# Autodesk Inventor assembly: Hand Assembly
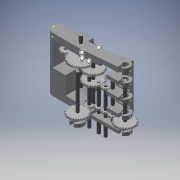
[picture p0: Inventor's stored thumbnail of the model, 180x180]
Saved by Autodesk Inventor 2017 (Build 210142000, 142)
## iProperties
Created: 2016-09-28
Part Number: Hand Assembly
Document SubType Name: Assembly
Designer: cmcdona
Author: cmcdona
## Documents named in this file (28)
- D:\julie\Documents\Cours McMaster\Graphics & Design\Project\Hand Assembly.iam
- D:\julie\Documents\Cours McMaster\Graphics & Design\Project\Hand - Frame.ipt
- D:\julie\Documents\Cours McMaster\Graphics & Design\Project\Hand - Digit 4.ipt
- D:\julie\Documents\Cours McMaster\Graphics & Design\Project\Hand - Digit 0-1.ipt
- D:\julie\Documents\Cours McMaster\Graphics & Design\Project\Hand - Distal Bridge.ipt
- D:\julie\Documents\Cours McMaster\Graphics & Design\Project\Hand - Digit 2-3.ipt
- D:\julie\Documents\Cours McMaster\Graphics & Design\Project\Hand - Proximal Bridge.ipt
- D:\julie\Documents\Cours McMaster\Graphics & Design\Project\Hand - Functional Workspace.ipt
- D:\julie\Documents\Cours McMaster\Graphics & Design\Project\Input Motor.ipt
- D:\julie\Documents\Cours McMaster\Graphics & Design\Project\Forefingers Rod.ipt
- D:\julie\Documents\Cours McMaster\Graphics & Design\Project\Hand Assembly\Design Accelerator\Spur Gears3.iam
- D:\julie\Documents\Cours McMaster\Graphics & Design\Project\Hand Assembly\Design Accelerator\Spur Gears4.iam
- D:\julie\Documents\Cours McMaster\Graphics & Design\Project\Hand Assembly\Design Accelerator\Spur Gears5.iam
- D:\julie\Documents\Cours McMaster\Graphics & Design\Project\Hand Assembly\Design Accelerator\Spur Gears6.iam
- D:\julie\Documents\Cours McMaster\Graphics & Design\Project\Hand Assembly\Design Accelerator\Spur Gear13.ipt
- D:\julie\Documents\Cours McMaster\Graphics & Design\Project\Hand Assembly\Design Accelerator\Spur Gear23.ipt
- D:\julie\Documents\Cours McMaster\Graphics & Design\Project\Hand Assembly\Design Accelerator\Spur Gear14.ipt
- D:\julie\Documents\Cours McMaster\Graphics & Design\Project\Hand Assembly\Design Accelerator\Spur Gear24.ipt
- D:\julie\Documents\Cours McMaster\Graphics & Design\Project\Hand Assembly\Design Accelerator\Spur Gear15.ipt
- D:\julie\Documents\Cours McMaster\Graphics & Design\Project\Hand Assembly\Design Accelerator\Spur Gear25.ipt
- D:\julie\Documents\Cours McMaster\Graphics & Design\Project\Hand Assembly\Design Accelerator\Spur Gear16.ipt
- D:\julie\Documents\Cours McMaster\Graphics & Design\Project\Hand Assembly\Design Accelerator\Spur Gear26.ipt
- D:\julie\Documents\Cours McMaster\Graphics & Design\Project\Hand Assembly\Design Accelerator\Spur Gears8.iam
- D:\julie\Documents\Cours McMaster\Graphics & Design\Project\Hand Assembly\Design Accelerator\Spur Gears9.iam
- D:\julie\Documents\Cours McMaster\Graphics & Design\Project\Hand Assembly\Design Accelerator\Spur Gear18.ipt
- D:\julie\Documents\Cours McMaster\Graphics & Design\Project\Hand Assembly\Design Accelerator\Spur Gear28.ipt
- D:\julie\Documents\Cours McMaster\Graphics & Design\Project\Hand Assembly\Design Accelerator\Spur Gear19.ipt
- D:\julie\Documents\Cours McMaster\Graphics & Design\Project\Hand Assembly\Design Accelerator\Spur Gear29.ipt
## Components (40 placed, 12 different names)
1. Hand - Frame:1 — Flush:1, Flush:2, Mate:1, Mate:2, Flush:3, Mate:3, Mate:16, Mate:17, Mate:18, Mate:22, Mate:23, Mate:25
2. Hand - Digit 4:1 — Flush:1, Flush:2, Mate:1, Mate:4, Mate:5, Mate:24
3. Hand - Digit 0-1:1 — Mate:2, Flush:3, Mate:3, Mate:6, Mate:19, Mate:20, Mate:21, Flush:4, Mate:37, Flush:23
4. Hand - Distal Bridge:1 — Mate:4, Mate:5, Mate:6, Mate:7, Mate:8, Mate:9, Mate:10, Mate:11, Mate:12, Mate:13, Mate:14, Mate:15
5. Hand - Digit 2-3:1 — Mate:7, Mate:8, Mate:9
6. Hand - Digit 2-3:2 — Mate:10, Mate:11, Mate:12
7. Hand - Digit 2-3:3 — Mate:13, Mate:14, Mate:15
8. Hand - Proximal Bridge:1 — Mate:16, Mate:17, Mate:18
9. Hand - Functional Workspace:1 — Mate:19, Mate:20, Mate:21
10. Input Motor:1 — Mate:22, Mate:23, Mate:25
11. Forefingers Rod:1 — Mate:24, Flush:4, Mate:26, Mate:27, Angle:1
12. Spur Gears:1 [sub-assembly]
13. Spur Gears:2 [sub-assembly]
14. Spur Gears:3 [sub-assembly]
15. Spur Gears:4 [sub-assembly]
16. Spur Gear1:1 — Mate:26, Flush:5
17. Spur Gear2:1 — Flush:5, Flush:6, Angle:1, Flush:10, Mate:39
18. Spur Gear1:2 — Flush:9, Flush:11, Mate:42
19. Spur Gear2:2 — Flush:9, Flush:11, Mate:41
20. Spur Gear1:3 — Flush:14, Mate:43
21. Spur Gear2:3 — Flush:14, Mate:36, Mate:44
22. Spur Gear1:4 — Mate:36, Flush:16, Mate:45
23. Spur Gear2:4 — Flush:16
24. Spur Gears:6 [sub-assembly]
25. Spur Gears:7 [sub-assembly]
26. Spur Gear1:5 — Flush:19
27. Spur Gear2:6 — Flush:18, Flush:19
28. Spur Gear1:6 — Flush:17, Flush:18
29. Spur Gear2:7 — Mate:27, Flush:17
30. Spur Gear2:8 — Flush:6, Flush:10, Flush:20, Flush:21, Mate:40
31. Spur Gear1:7 — Flush:20, Mate:38
32. Spur Gear2:9 — Flush:21, Flush:22, Mate:46
33. Spur Gear2:10 — Flush:22, Mate:47
34. Forefingers Rod:2 — Mate:39
35. Forefingers Rod:3 — Mate:37, Flush:23, Mate:38
36. Forefingers Rod:4 — Mate:40, Mate:41
37. Forefingers Rod:5 — Mate:42, Mate:43
38. Forefingers Rod:6 — Mate:44, Mate:45
39. Forefingers Rod:7 — Mate:46
40. Forefingers Rod:8 — Mate:47
## Relationships (58: Mate 39, Flush 18, Angle 1)
- Flush:1: Hand - Frame:1 ↔ Hand - Digit 4:1
- Flush:2: Hand - Frame:1 ↔ Hand - Digit 4:1
- Mate:1: Hand - Frame:1 ↔ Hand - Digit 4:1
- Mate:2: Hand - Frame:1 ↔ Hand - Digit 0-1:1
- Flush:3: Hand - Frame:1 ↔ Hand - Digit 0-1:1
- Mate:3: Hand - Frame:1 ↔ Hand - Digit 0-1:1
- Mate:4: Hand - Digit 4:1 ↔ Hand - Distal Bridge:1
- Mate:5: Hand - Digit 4:1 ↔ Hand - Distal Bridge:1
- Mate:6: Hand - Digit 0-1:1 ↔ Hand - Distal Bridge:1
- Mate:7: Hand - Distal Bridge:1 ↔ Hand - Digit 2-3:1
- Mate:8: Hand - Distal Bridge:1 ↔ Hand - Digit 2-3:1
- Mate:9: Hand - Distal Bridge:1 ↔ Hand - Digit 2-3:1
- Mate:10: Hand - Distal Bridge:1 ↔ Hand - Digit 2-3:2
- Mate:11: Hand - Distal Bridge:1 ↔ Hand - Digit 2-3:2
- Mate:12: Hand - Distal Bridge:1 ↔ Hand - Digit 2-3:2
- Mate:13: Hand - Distal Bridge:1 ↔ Hand - Digit 2-3:3
- Mate:14: Hand - Distal Bridge:1 ↔ Hand - Digit 2-3:3
- Mate:15: Hand - Distal Bridge:1 ↔ Hand - Digit 2-3:3
- Mate:16: Hand - Frame:1 ↔ Hand - Proximal Bridge:1
- Mate:17: Hand - Frame:1 ↔ Hand - Proximal Bridge:1
- Mate:18: Hand - Frame:1 ↔ Hand - Proximal Bridge:1
- Mate:19: Hand - Digit 0-1:1 ↔ Hand - Functional Workspace:1
- Mate:20 (41 mm): Hand - Digit 0-1:1 ↔ Hand - Functional Workspace:1
- Mate:21 (33 mm): Hand - Digit 0-1:1 ↔ Hand - Functional Workspace:1
- Mate:22: Hand - Frame:1 ↔ Input Motor:1
- Mate:23: Hand - Frame:1 ↔ Input Motor:1
- Mate:24: Hand - Digit 4:1 ↔ Forefingers Rod:1
- Flush:4: Hand - Digit 0-1:1 ↔ Forefingers Rod:1
- Mate:25 (6 mm): Hand - Frame:1 ↔ Input Motor:1
- Mate:26: Forefingers Rod:1 ↔ Spur Gear1:1
- Flush:5: Spur Gear1:1 ↔ Spur Gear2:1
- Mate:27: Forefingers Rod:1 ↔ Spur Gear2:7
- Flush:6: Spur Gear2:1 ↔ Spur Gear2:8
- Angle:1 (0 deg): Forefingers Rod:1 ↔ Spur Gear2:1
- Flush:9: Spur Gear1:2 ↔ Spur Gear2:2
- Flush:10: Spur Gear2:1 ↔ Spur Gear2:8
- Flush:11: Spur Gear1:2 ↔ Spur Gear2:2
- Flush:14: Spur Gear1:3 ↔ Spur Gear2:3
- Mate:36: Spur Gear2:3 ↔ Spur Gear1:4
- Flush:16: Spur Gear1:4 ↔ Spur Gear2:4
- Flush:17: Spur Gear1:6 ↔ Spur Gear2:7
- Flush:18: Spur Gear2:6 ↔ Spur Gear1:6
- Flush:19: Spur Gear1:5 ↔ Spur Gear2:6
- Flush:20: Spur Gear2:8 ↔ Spur Gear1:7
- Flush:21: Spur Gear2:8 ↔ Spur Gear2:9
- Flush:22: Spur Gear2:9 ↔ Spur Gear2:10
- Mate:37: Hand - Digit 0-1:1 ↔ Forefingers Rod:3
- Flush:23: Hand - Digit 0-1:1 ↔ Forefingers Rod:3
- Mate:38: Spur Gear1:7 ↔ Forefingers Rod:3
- Mate:39: Spur Gear2:1 ↔ Forefingers Rod:2
- Mate:40: Spur Gear2:8 ↔ Forefingers Rod:4
- Mate:41: Spur Gear2:2 ↔ Forefingers Rod:4
- Mate:42: Spur Gear1:2 ↔ Forefingers Rod:5
- Mate:43: Spur Gear1:3 ↔ Forefingers Rod:5
- Mate:44: Spur Gear2:3 ↔ Forefingers Rod:6
- Mate:45: Spur Gear1:4 ↔ Forefingers Rod:6
- Mate:46: Spur Gear2:9 ↔ Forefingers Rod:7
- Mate:47: Spur Gear2:10 ↔ Forefingers Rod:8
